# Autodesk Inventor assembly: CyberOrto
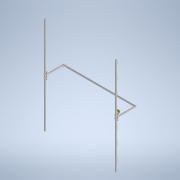
[picture p0: Inventor's stored thumbnail of the model, 180x180]
Saved by Autodesk Inventor 2022 (Build 260153000, 153)
## iProperties
RuleStatus: InUse
Created: 2021-12-29
Part Number: CyberOrto
Document SubType Name: Assembly
Designer: matte
Author: matte
## Documents named in this file (21)
- C:\Users\Elia\Documents\ELIA\UNITN\MAGISTRALE\1st year\1st semester\Mechanical Design\Project\MDM-CyberOrto-CAD-main\CyberOrto.iam
- C:\Users\Elia\Documents\ELIA\UNITN\MAGISTRALE\1st year\1st semester\Mechanical Design\Project\MDM-CyberOrto-CAD-main\Pezzi singoli\Trave Principale.ipt
- C:\Users\Elia\Documents\ELIA\UNITN\MAGISTRALE\1st year\1st semester\Mechanical Design\Project\MDM-CyberOrto-CAD-main\Pezzi singoli\Supporto SX.ipt
- C:\Users\Elia\Documents\ELIA\UNITN\MAGISTRALE\1st year\1st semester\Mechanical Design\Project\MDM-CyberOrto-CAD-main\Parker components\03-Brackets_Gussets_Plates\09-Machined Gussets\20-102.ipt
- C:\Users\Elia\Documents\ELIA\UNITN\MAGISTRALE\1st year\1st semester\Mechanical Design\Project\MDM-CyberOrto-CAD-main\Parker components\02-Fasteners\10-Standard T-Nuts\20-050.ipt
- C:\Users\Elia\Documents\ELIA\UNITN\MAGISTRALE\1st year\1st semester\Mechanical Design\Project\MDM-CyberOrto-CAD-main\Parker components\02-Fasteners\16-Screws\01-Metric Screws\01-Button Head\24-118-8.ipt
- C:\Users\Elia\Documents\ELIA\UNITN\MAGISTRALE\1st year\1st semester\Mechanical Design\Project\MDM-CyberOrto-CAD-main\Guida a terra.iam
- C:\Users\Elia\Documents\ELIA\UNITN\MAGISTRALE\1st year\1st semester\Mechanical Design\Project\MDM-CyberOrto-CAD-main\Parker components\05-Handles_Hinges\13-Pivot Joints\23-010.iam
- C:\Users\Elia\Documents\ELIA\UNITN\MAGISTRALE\1st year\1st semester\Mechanical Design\Project\MDM-CyberOrto-CAD-main\Parker components\02-Fasteners\10-Standard T-Nuts\20-058.ipt
- C:\Users\Elia\Documents\ELIA\UNITN\MAGISTRALE\1st year\1st semester\Mechanical Design\Project\MDM-CyberOrto-CAD-main\Parker components\02-Fasteners\16-Screws\01-Metric Screws\01-Button Head\24-116-8.ipt
- C:\Users\Elia\Documents\ELIA\UNITN\MAGISTRALE\1st year\1st semester\Mechanical Design\Project\MDM-CyberOrto-CAD-main\Pezzi singoli\Supporto DX.ipt
- C:\Users\Elia\Documents\ELIA\UNITN\MAGISTRALE\1st year\1st semester\Mechanical Design\Project\MDM-CyberOrto-CAD-main\Parker components\02-Fasteners\16-Screws\01-Metric Screws\01-Button Head\24-120-8.ipt
- C:\Users\Elia\Documents\ELIA\UNITN\MAGISTRALE\1st year\1st semester\Mechanical Design\Project\MDM-CyberOrto-CAD-main\Pezzi singoli\Supporto lineare\Carrello semplice.iam
- C:\Users\Elia\Documents\ELIA\UNITN\MAGISTRALE\1st year\1st semester\Mechanical Design\Project\MDM-CyberOrto-CAD-main\Pezzi singoli\Pista Orizzontale.iam
- C:\Users\Elia\Documents\ELIA\UNITN\MAGISTRALE\1st year\1st semester\Mechanical Design\Project\MDM-CyberOrto-CAD-main\Platform.ipt
- C:\Users\Elia\Documents\ELIA\UNITN\MAGISTRALE\1st year\1st semester\Mechanical Design\Project\MDM-CyberOrto-CAD-main\Parker components\02-Fasteners\16-Screws\01-Metric Screws\01-Button Head\24-130-6.ipt
- C:\Users\Elia\Documents\ELIA\UNITN\MAGISTRALE\1st year\1st semester\Mechanical Design\Project\MDM-CyberOrto-CAD-main\Parker components\02-Fasteners\15-T-Bolts_Nuts_Washers\03-Washers\24-700-6.ipt
- C:\Users\Elia\Documents\ELIA\UNITN\MAGISTRALE\1st year\1st semester\Mechanical Design\Project\MDM-CyberOrto-CAD-main\Parker components\02-Fasteners\15-T-Bolts_Nuts_Washers\02-Nuts\24-706-6.ipt
- C:\Users\Elia\Documents\ELIA\UNITN\MAGISTRALE\1st year\1st semester\Mechanical Design\Project\MDM-CyberOrto-CAD-main\Servo Motor 50W\bch2mba531ca5c.ipt
- C:\Users\Elia\Documents\ELIA\UNITN\MAGISTRALE\1st year\1st semester\Mechanical Design\Project\MDM-CyberOrto-CAD-main\Rack_Pinion\Rack gear scaled1.ipt
- C:\Users\Elia\Documents\ELIA\UNITN\MAGISTRALE\1st year\1st semester\Mechanical Design\Project\MDM-CyberOrto-CAD-main\Rack_Pinion\pinion_scaled1.ipt
## Components (59 placed, 20 different names)
1. Trave Principale:1 — Coincidente:1, Coincidente:2, Coincidente:3, Allineato:1, Coincidente:4, Allineato:2, Coincidente:5, Coincidente:10, Coincidente:40, Allineato:5, Allineato:6, Coincidente:41, Angolo:1
2. Supporto SX:1 — Allineato:1, Coincidente:4, Allineato:2, Coincidente:6, Allineato:3, Coincidente:7, Coincidente:15, Coincidente:16, Coincidente:23, Coincidente:28, Coincidente:29, Coincidente:30
3. Supporto DX:1 — Coincidente:45, Allineato:7, Allineato:8, Coincidente:48, Allineato:9, Allineato:10
4. 24-118-8:3 — Coincidente:19, Coincidente:20
5. 24-118-8:4 — Coincidente:21, Coincidente:22
6. 20-050:2 — Coincidente:10, Coincidente:11, Coincidente:12
7. 24-118-8:1 — Coincidente:13, Coincidente:14
8. 24-118-8:2 — Coincidente:17, Coincidente:18
9. 20-102:1 — Coincidente:5, Coincidente:6, Allineato:3, Coincidente:8, Coincidente:9, Coincidente:11, Coincidente:12, Coincidente:13, Coincidente:14, Coincidente:17, Coincidente:18, Coincidente:19, Coincidente:20, Coincidente:21, Coincidente:22
10. 20-050:1 — Coincidente:7, Coincidente:8, Coincidente:9
11. 24-118-8:5 — Coincidente:31, Coincidente:32, Coincidente:33
12. 24-118-8:6 — Coincidente:34, Coincidente:35
13. 24-118-8:7 — Coincidente:38, Coincidente:39
14. 24-118-8:8 — Coincidente:36, Coincidente:37
15. Guida a terra:1 [sub-assembly] — Coincidente:15, Coincidente:16, Coincidente:23, Coincidente:32, Coincidente:33, Coincidente:34, Coincidente:35, Coincidente:36, Coincidente:37, Coincidente:38, Coincidente:39, Allineato:12
16. 20-050:3 — Coincidente:27, Allineato:4, Coincidente:28, Coincidente:30, Coincidente:31
17. 20-050:4 — Coincidente:27, Allineato:4, Coincidente:29
18. 23-010:1 [sub-assembly] — Coincidente:40, Allineato:5, Allineato:6, Coincidente:43, Coincidente:44, Coincidente:45, Allineato:7, Allineato:8, Coincidente:46, Coincidente:47
19. 20-058:1 — Coincidente:41, Angolo:1, Coincidente:42
20. 24-116-8:1 — Coincidente:42, Coincidente:43, Coincidente:44
21. 24-120-8:1 — Coincidente:46, Coincidente:47
22. 24-120-8:2 — Coincidente:51, Coincidente:52
23. Carrello semplice:1 [sub-assembly] — Coincidente:48, Allineato:9, Allineato:10, Coincidente:49, Allineato:11, Coincidente:51, Coincidente:52, Coincidente:53, Allineato:13, Coincidente:54, Coincidente:56, Coincidente:58, Coincidente:60, Coincidente:62
24. Pista Orizzontale:1 [sub-assembly] — Coincidente:49, Allineato:11, Allineato:12, Coincidente:72, Coincidente:73, Coincidente:76, Coincidente:78, Coincidente:79, Coincidente:81, Coincidente:85, Coincidente:87, Coincidente:88, Coincidente:90, Coincidente:93, Coincidente:95, Coincidente:96, Coincidente:99, Coincidente:100, Coincidente:103, Coincidente:104, Coincidente:107, Allineato:32, Coincidente:110, Coincidente:112
25. 24-130-6:1 — Inserimento:1, Coincidente:61
26. 24-700-6:1 — Inserimento:1, Inserimento:7
27. 24-706-6:1 — Coincidente:55, Coincidente:56
28. 24-130-6:2 — Coincidente:59
29. 24-700-6:3 — Inserimento:6
30. 24-130-6:3 — Coincidente:57
31. 24-700-6:2 — Inserimento:8
32. 24-130-6:4 — Coincidente:55
33. 24-700-6:4 — Inserimento:5
34. 24-706-6:2 — Coincidente:57, Coincidente:58
35. 24-706-6:3 — Coincidente:61, Coincidente:62
36. 24-706-6:4 — Coincidente:59, Coincidente:60
37. Platform:1 — Coincidente:53, Allineato:13, Coincidente:54, Inserimento:5, Inserimento:6, Inserimento:7, Inserimento:8, Coincidente:63, Coincidente:64, Coincidente:65, Coincidente:66, Coincidente:67, Coincidente:68
38. bch2mba531ca5c:1 — Coincidente:66, Coincidente:67, Coincidente:68, Coincidente:113
39. Rack gear scaled1:4 — Coincidente:72, Coincidente:74, Allineato:15, Coincidente:108, Allineato:33
40. Rack gear scaled1:5 — Coincidente:77, Allineato:17, Coincidente:78, Allineato:18, Coincidente:80
41. Rack gear scaled1:6 — Coincidente:75, Coincidente:76, Allineato:16, Coincidente:77, Allineato:17
42. Rack gear scaled1:7 — Allineato:19, Coincidente:81, Coincidente:82, Allineato:20, Coincidente:83
43. Rack gear scaled1:8 — Coincidente:73, Coincidente:74, Allineato:15, Coincidente:75, Allineato:16
44. Rack gear scaled1:9 — Coincidente:79, Allineato:18, Coincidente:80, Allineato:19, Coincidente:82
45. Rack gear scaled1:10 — Coincidente:86, Coincidente:87, Allineato:21, Coincidente:89, Allineato:22
46. Rack gear scaled1:11 — Allineato:20, Coincidente:83, Coincidente:85, Coincidente:86, Allineato:21
47. Rack gear scaled1:12 — Coincidente:92, Coincidente:93, Allineato:24, Coincidente:94, Allineato:25
48. Rack gear scaled1:13 — Coincidente:88, Coincidente:89, Allineato:22, Allineato:32
49. Rack gear scaled1:14 — Coincidente:90, Coincidente:92, Allineato:24, Coincidente:108, Allineato:33, Allineato:36, Allineato:37
50. Rack gear scaled1:15 — Coincidente:94, Coincidente:95, Allineato:25, Coincidente:97, Allineato:26
51. Rack gear scaled1:16 — Coincidente:96, Coincidente:97, Allineato:26, Coincidente:98, Allineato:27
52. Rack gear scaled1:17 — Coincidente:98, Coincidente:99, Allineato:27, Coincidente:101, Allineato:28
53. Rack gear scaled1:19 — Coincidente:104, Coincidente:105, Allineato:30, Coincidente:106, Allineato:31
54. Rack gear scaled1:20 — Coincidente:102, Coincidente:103, Allineato:29, Coincidente:105, Allineato:30
55. Rack gear scaled1:18 — Coincidente:100, Coincidente:101, Allineato:28, Coincidente:102, Allineato:29
56. Rack gear scaled1:21 — Coincidente:106, Coincidente:107, Allineato:31, Coincidente:109, Allineato:34
57. Rack gear scaled1:22 — Coincidente:109, Coincidente:110, Allineato:34, Coincidente:111, Allineato:35
58. Rack gear scaled1:23 — Coincidente:111, Coincidente:112, Allineato:35
59. pinion_scaled1:1 — Coincidente:113, Allineato:36, Tangente:1
## Relationships (149: Mate 104, Flush 35, Insert 8, Angle 1, Tangent 1)
- Coincidente:1 [Mate]: Trave Principale:1
- Coincidente:2 [Mate]: Trave Principale:1
- Coincidente:3 [Mate]: Trave Principale:1
- Allineato:1 [Flush]: Trave Principale:1 ↔ Supporto SX:1
- Coincidente:4 [Mate]: Trave Principale:1 ↔ Supporto SX:1
- Allineato:2 [Flush]: Trave Principale:1 ↔ Supporto SX:1
- Coincidente:5 [Mate]: Trave Principale:1 ↔ 20-102:1
- Coincidente:6 [Mate]: Supporto SX:1 ↔ 20-102:1
- Allineato:3 [Flush]: Supporto SX:1 ↔ 20-102:1
- Coincidente:7 [Mate]: Supporto SX:1 ↔ 20-050:1
- Coincidente:8 [Mate]: 20-102:1 ↔ 20-050:1
- Coincidente:9 [Mate]: 20-102:1 ↔ 20-050:1
- Coincidente:10 [Mate]: Trave Principale:1 ↔ 20-050:2
- Coincidente:11 [Mate]: 20-050:2 ↔ 20-102:1
- Coincidente:12 [Mate]: 20-050:2 ↔ 20-102:1
- Coincidente:13 [Mate]: 24-118-8:1 ↔ 20-102:1
- Coincidente:14 [Mate]: 24-118-8:1 ↔ 20-102:1
- Coincidente:15 [Mate]: Supporto SX:1 ↔ Guida a terra:1
- Coincidente:16 [Mate]: Supporto SX:1 ↔ Guida a terra:1
- Coincidente:17 [Mate]: 24-118-8:2 ↔ 20-102:1
- Coincidente:18 [Mate]: 24-118-8:2 ↔ 20-102:1
- Coincidente:19 [Mate]: 24-118-8:3 ↔ 20-102:1
- Coincidente:20 [Mate]: 24-118-8:3 ↔ 20-102:1
- Coincidente:21 [Mate]: 24-118-8:4 ↔ 20-102:1
- Coincidente:22 [Mate]: 24-118-8:4 ↔ 20-102:1
- Coincidente:23 [Mate]: Supporto SX:1 ↔ Guida a terra:1
- Coincidente:27 [Mate]: 20-050:3 ↔ 20-050:4
- Allineato:4 [Flush]: 20-050:3 ↔ 20-050:4
- Coincidente:28 [Mate]: Supporto SX:1 ↔ 20-050:3
- Coincidente:29 [Mate]: Supporto SX:1 ↔ 20-050:4
- Coincidente:30 [Mate]: Supporto SX:1 ↔ 20-050:3
- Coincidente:31 [Mate]: 24-118-8:5 ↔ 20-050:3
- Coincidente:32 [Mate]: 24-118-8:5 ↔ Guida a terra:1
- Coincidente:33 [Mate]: 24-118-8:5 ↔ Guida a terra:1
- Coincidente:34 [Mate]: 24-118-8:6 ↔ Guida a terra:1
- Coincidente:35 [Mate]: 24-118-8:6 ↔ Guida a terra:1
- Coincidente:36 [Mate]: 24-118-8:8 ↔ Guida a terra:1
- Coincidente:37 [Mate]: 24-118-8:8 ↔ Guida a terra:1
- Coincidente:38 [Mate]: 24-118-8:7 ↔ Guida a terra:1
- Coincidente:39 [Mate]: 24-118-8:7 ↔ Guida a terra:1
- Coincidente:40 [Mate]: Trave Principale:1 ↔ 23-010:1
- Allineato:5 [Flush]: Trave Principale:1 ↔ 23-010:1
- Allineato:6 [Flush]: Trave Principale:1 ↔ 23-010:1
- Coincidente:41 [Mate]: Trave Principale:1 ↔ 20-058:1
- Angolo:1 [Angle] (0 deg): Trave Principale:1 ↔ 20-058:1
- Coincidente:42 [Mate]: 20-058:1 ↔ 24-116-8:1
- Coincidente:43 [Mate]: 23-010:1 ↔ 24-116-8:1
- Coincidente:44 [Mate]: 23-010:1 ↔ 24-116-8:1
- Coincidente:45 [Mate]: Supporto DX:1 ↔ 23-010:1
- Allineato:7 [Flush]: Supporto DX:1 ↔ 23-010:1
- Allineato:8 [Flush]: Supporto DX:1 ↔ 23-010:1
- Coincidente:46 [Mate]: 23-010:1 ↔ 24-120-8:1
- Coincidente:47 [Mate]: 23-010:1 ↔ 24-120-8:1
- Coincidente:48 [Mate]: Supporto DX:1 ↔ Carrello semplice:1
- Allineato:9 [Flush]: Supporto DX:1 ↔ Carrello semplice:1
- Allineato:10 [Flush]: Supporto DX:1 ↔ Carrello semplice:1
- Coincidente:49 [Mate] (20 mm): Carrello semplice:1 ↔ Pista Orizzontale:1
- Allineato:11 [Flush] (20 mm): Carrello semplice:1 ↔ Pista Orizzontale:1
- Allineato:12 [Flush]: Guida a terra:1 ↔ Pista Orizzontale:1
- Coincidente:51 [Mate]: 24-120-8:2 ↔ Carrello semplice:1
- Coincidente:52 [Mate]: 24-120-8:2 ↔ Carrello semplice:1
- Coincidente:53 [Mate]: Carrello semplice:1 ↔ Platform:1
- Allineato:13 [Flush]: Carrello semplice:1 ↔ Platform:1
- Coincidente:54 [Mate]: Carrello semplice:1 ↔ Platform:1
- Inserimento:1: 24-130-6:1 ↔ 24-700-6:1
- [Insert]: 24-130-6:2 ↔ 24-700-6:2
- [Insert]: 24-700-6:3 ↔ 24-130-6:3
- [Insert]: 24-130-6:4 ↔ 24-700-6:4
- Inserimento:5: 24-700-6:4 ↔ Platform:1
- Inserimento:6: 24-700-6:3 ↔ Platform:1
- Inserimento:7: 24-700-6:1 ↔ Platform:1
- Inserimento:8: 24-700-6:2 ↔ Platform:1
- Coincidente:55 [Mate]: 24-706-6:1 ↔ 24-130-6:4
- Coincidente:56 [Mate]: Carrello semplice:1 ↔ 24-706-6:1
- Coincidente:57 [Mate]: 24-130-6:3 ↔ 24-706-6:2
- Coincidente:58 [Mate]: Carrello semplice:1 ↔ 24-706-6:2
- Coincidente:59 [Mate]: 24-130-6:2 ↔ 24-706-6:4
- Coincidente:60 [Mate]: Carrello semplice:1 ↔ 24-706-6:4
- Coincidente:61 [Mate]: 24-130-6:1 ↔ 24-706-6:3
- Coincidente:62 [Mate]: Carrello semplice:1 ↔ 24-706-6:3
- Coincidente:63 [Mate]: Platform:1
- Coincidente:64 [Mate]: Platform:1
- Coincidente:65 [Mate]: Platform:1
- Coincidente:66 [Mate]: Platform:1 ↔ bch2mba531ca5c:1
- Coincidente:67 [Mate]: Platform:1 ↔ bch2mba531ca5c:1
- Coincidente:68 [Mate]: Platform:1 ↔ bch2mba531ca5c:1
- Coincidente:72 [Mate]: Pista Orizzontale:1 ↔ Rack gear scaled1:4
- Coincidente:73 [Mate]: Pista Orizzontale:1 ↔ Rack gear scaled1:8
- Coincidente:74 [Mate]: Rack gear scaled1:4 ↔ Rack gear scaled1:8
- Allineato:15 [Flush]: Rack gear scaled1:4 ↔ Rack gear scaled1:8
- Coincidente:75 [Mate]: Rack gear scaled1:6 ↔ Rack gear scaled1:8
- Coincidente:76 [Mate]: Pista Orizzontale:1 ↔ Rack gear scaled1:6
- Allineato:16 [Flush]: Rack gear scaled1:6 ↔ Rack gear scaled1:8
- Coincidente:77 [Mate]: Rack gear scaled1:5 ↔ Rack gear scaled1:6
- Allineato:17 [Flush]: Rack gear scaled1:5 ↔ Rack gear scaled1:6
- Coincidente:78 [Mate]: Pista Orizzontale:1 ↔ Rack gear scaled1:5
- Coincidente:79 [Mate]: Pista Orizzontale:1 ↔ Rack gear scaled1:9
- Allineato:18 [Flush]: Rack gear scaled1:5 ↔ Rack gear scaled1:9
- Coincidente:80 [Mate]: Rack gear scaled1:5 ↔ Rack gear scaled1:9
- Allineato:19 [Flush]: Rack gear scaled1:7 ↔ Rack gear scaled1:9
- Coincidente:81 [Mate]: Pista Orizzontale:1 ↔ Rack gear scaled1:7
- Coincidente:82 [Mate]: Rack gear scaled1:7 ↔ Rack gear scaled1:9
- Allineato:20 [Flush]: Rack gear scaled1:7 ↔ Rack gear scaled1:11
- Coincidente:83 [Mate]: Rack gear scaled1:7 ↔ Rack gear scaled1:11
- Coincidente:85 [Mate]: Pista Orizzontale:1 ↔ Rack gear scaled1:11
- Coincidente:86 [Mate]: Rack gear scaled1:10 ↔ Rack gear scaled1:11
- Coincidente:87 [Mate]: Pista Orizzontale:1 ↔ Rack gear scaled1:10
- Allineato:21 [Flush]: Rack gear scaled1:10 ↔ Rack gear scaled1:11
- Coincidente:88 [Mate]: Pista Orizzontale:1 ↔ Rack gear scaled1:13
- Coincidente:89 [Mate]: Rack gear scaled1:10 ↔ Rack gear scaled1:13
- Allineato:22 [Flush]: Rack gear scaled1:10 ↔ Rack gear scaled1:13
- Coincidente:90 [Mate]: Pista Orizzontale:1 ↔ Rack gear scaled1:14
- Coincidente:92 [Mate]: Rack gear scaled1:12 ↔ Rack gear scaled1:14
- Coincidente:93 [Mate]: Pista Orizzontale:1 ↔ Rack gear scaled1:12
- Allineato:24 [Flush]: Rack gear scaled1:12 ↔ Rack gear scaled1:14
- Coincidente:94 [Mate]: Rack gear scaled1:12 ↔ Rack gear scaled1:15
- Coincidente:95 [Mate]: Pista Orizzontale:1 ↔ Rack gear scaled1:15
- Allineato:25 [Flush]: Rack gear scaled1:12 ↔ Rack gear scaled1:15
- Coincidente:96 [Mate]: Pista Orizzontale:1 ↔ Rack gear scaled1:16
- Coincidente:97 [Mate]: Rack gear scaled1:15 ↔ Rack gear scaled1:16
- Allineato:26 [Flush]: Rack gear scaled1:15 ↔ Rack gear scaled1:16
- Coincidente:98 [Mate]: Rack gear scaled1:16 ↔ Rack gear scaled1:17
- Coincidente:99 [Mate]: Pista Orizzontale:1 ↔ Rack gear scaled1:17
- Allineato:27 [Flush]: Rack gear scaled1:16 ↔ Rack gear scaled1:17
- Coincidente:100 [Mate]: Pista Orizzontale:1 ↔ Rack gear scaled1:18
- Coincidente:101 [Mate]: Rack gear scaled1:17 ↔ Rack gear scaled1:18
- Allineato:28 [Flush]: Rack gear scaled1:17 ↔ Rack gear scaled1:18
- Coincidente:102 [Mate]: Rack gear scaled1:20 ↔ Rack gear scaled1:18
- Coincidente:103 [Mate]: Pista Orizzontale:1 ↔ Rack gear scaled1:20
- Allineato:29 [Flush]: Rack gear scaled1:20 ↔ Rack gear scaled1:18
- Coincidente:104 [Mate]: Pista Orizzontale:1 ↔ Rack gear scaled1:19
- Coincidente:105 [Mate]: Rack gear scaled1:19 ↔ Rack gear scaled1:20
- Allineato:30 [Flush]: Rack gear scaled1:19 ↔ Rack gear scaled1:20
- Coincidente:106 [Mate]: Rack gear scaled1:19 ↔ Rack gear scaled1:21
- Coincidente:107 [Mate]: Pista Orizzontale:1 ↔ Rack gear scaled1:21
- Allineato:31 [Flush]: Rack gear scaled1:19 ↔ Rack gear scaled1:21
- Allineato:32 [Flush]: Pista Orizzontale:1 ↔ Rack gear scaled1:13
- Coincidente:108 [Mate]: Rack gear scaled1:4 ↔ Rack gear scaled1:14
- Allineato:33 [Flush]: Rack gear scaled1:4 ↔ Rack gear scaled1:14
- Coincidente:109 [Mate]: Rack gear scaled1:21 ↔ Rack gear scaled1:22
- Coincidente:110 [Mate]: Pista Orizzontale:1 ↔ Rack gear scaled1:22
- Allineato:34 [Flush]: Rack gear scaled1:21 ↔ Rack gear scaled1:22
- Coincidente:111 [Mate]: Rack gear scaled1:22 ↔ Rack gear scaled1:23
- Coincidente:112 [Mate]: Pista Orizzontale:1 ↔ Rack gear scaled1:23
- Allineato:35 [Flush]: Rack gear scaled1:22 ↔ Rack gear scaled1:23
- Coincidente:113 [Mate]: bch2mba531ca5c:1 ↔ pinion_scaled1:1
- Allineato:36 [Flush]: Rack gear scaled1:14 ↔ pinion_scaled1:1
- Allineato:37 [Flush] (-0.9524 mm): Rack gear scaled1:14
- Tangente:1: pinion_scaled1:1
## Named parameters: L_piatto_guide = 240 mm, L_tracce_terra = 4000 mm, L_traccia_superiore = 3000 mm, H_supporto = 700 mm, d116_d115 = 0 mm, d117_d115 = 0 mm, d118_d115 = 0 mm
